# Autodesk Inventor assembly: bett_V2_sitzbank_mit_deckel
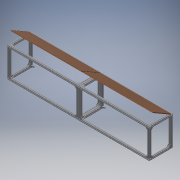
[picture p0: Inventor's stored thumbnail of the model, 180x180]
Saved by Autodesk Inventor 2018 (Build 220112000, 112)
## iProperties
Created: 2020-04-13
Part Number: bett_V2_sitzbank_mit_deckel
Material: Generisch
Document SubType Name: Assembly
Designer: wepet
Author: wepet
## Documents named in this file (3)
- C:\Users\wepet\Downloads\anhaenger\current\details\bett\bett_V2_sitzbank_mit_deckel.iam
- C:\Users\wepet\Downloads\anhaenger\current\details\bett\bett_V2_deckplatte.ipt
- C:\Users\wepet\Downloads\anhaenger\current\details\bett\bett_V2_sitzbank.iam
## Components (4 placed, 2 different names)
1. bett_V2_deckplatte:1 — Drehbar:1
2. bett_V2_sitzbank:1 [sub-assembly] — Passend:1, Passend:2, Fluchtend:1, Passend:3, Fluchtend:2, Fluchtend:3, Drehbar:1
3. bett_V2_sitzbank:2 [sub-assembly] — Passend:3, Fluchtend:2, Fluchtend:3, Drehbar:2
4. bett_V2_deckplatte:2 — Drehbar:2
## Relationships (8: Mate 3, Flush 3, RevoluteJoint 2)
- Passend:1 [Mate]: bett_V2_sitzbank:1
- Passend:2 [Mate]: bett_V2_sitzbank:1
- Fluchtend:1 [Flush]: bett_V2_sitzbank:1
- Passend:3 [Mate]: bett_V2_sitzbank:1 ↔ bett_V2_sitzbank:2
- Fluchtend:2 [Flush]: bett_V2_sitzbank:1 ↔ bett_V2_sitzbank:2
- Fluchtend:3 [Flush]: bett_V2_sitzbank:1 ↔ bett_V2_sitzbank:2
- Drehbar:1 [RevoluteJoint]: bett_V2_deckplatte:1 ↔ bett_V2_sitzbank:1
- Drehbar:2 [RevoluteJoint]: bett_V2_sitzbank:2 ↔ bett_V2_deckplatte:2
